# Autodesk Inventor assembly: E005_Boitier_v3
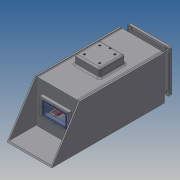
[picture p0: Inventor's stored thumbnail of the model, 180x180]
Saved by Autodesk Inventor 2021.3 (Build 253353000, 353)
## iProperties
Created: 2021-11-26
Part Number: E005_Boitier_v3
Document SubType Name: Assembly
Designer: gabri
Author: gabri
## Documents named in this file (6)
- D:\PGA\E005_Boitier_v3.iam
- D:\PGA\P033_Boitier_v3.ipt
- D:\PGA\E003_BoitierEcran.iam
- D:\PGA\P034_Casquette.ipt
- D:\PGA\P016_FondBoitierCapteurs.ipt
- D:\PGA\P035_FondBoitierv3.ipt
## Components (5 placed, 5 different names)
1. P033_Boitier_v3:1 — Mate:1, Mate:2, Mate:3, Flush:1, Mate:4, Mate:5, Mate:6, Mate:7, Mate:8, Mate:10, Mate:11, Flush:2
2. E003_BoitierEcran:1 [sub-assembly] — Flush:1, Mate:4, Mate:5
3. P034_Casquette:1 — Mate:6, Mate:7, Flush:2
4. P016_FondBoitierCapteurs:1 — Mate:8
5. P035_FondBoitierv3:1 — Mate:10, Mate:11
## Relationships (12: Mate 10, Flush 2)
- Mate:1: P033_Boitier_v3:1
- Mate:2: P033_Boitier_v3:1
- Mate:3: P033_Boitier_v3:1
- Flush:1: P033_Boitier_v3:1 ↔ E003_BoitierEcran:1
- Mate:4: P033_Boitier_v3:1 ↔ E003_BoitierEcran:1
- Mate:5: P033_Boitier_v3:1 ↔ E003_BoitierEcran:1
- Mate:6: P033_Boitier_v3:1 ↔ P034_Casquette:1
- Mate:7: P033_Boitier_v3:1 ↔ P034_Casquette:1
- Mate:8: P033_Boitier_v3:1 ↔ P016_FondBoitierCapteurs:1
- Mate:10: P033_Boitier_v3:1 ↔ P035_FondBoitierv3:1
- Mate:11: P033_Boitier_v3:1 ↔ P035_FondBoitierv3:1
- Flush:2: P033_Boitier_v3:1 ↔ P034_Casquette:1
